# Autodesk Inventor assembly: cubi
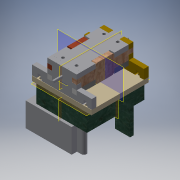
[picture p0: Inventor's stored thumbnail of the model, 180x180]
Saved by Autodesk Inventor 2018 (Build 220112000, 112)
## iProperties
Created: 2018-07-19
Part Number: cubi
Document SubType Name: Assembly
Designer: julien.allali
Author: julien.allali
## Documents named in this file (6)
- C:\Users\julien.allali\Documents\cubi\cubi.iam
- C:\Users\julien.allali\Documents\moteur.ipt
- C:\Users\julien.allali\Documents\cubi\board.ipt
- C:\Users\julien.allali\Documents\cubi\bat9V.ipt
- C:\Users\julien.allali\Documents\cubi\connector9V.ipt
- C:\Users\julien.allali\Documents\cubi\box.ipt
## Components (6 placed, 5 different names)
1. moteur:1 — Flush:1, Mate:1, Flush:2, Symmetry:1, Symmetry:2, Flush:5
2. moteur:2 — Flush:1, Mate:1, Flush:2, Mate:3, Symmetry:1, Symmetry:2, Flush:6
3. board:1 — Mate:2, Rotational:1, Mate:3, Mate:4, Mate:5, Flush:4, Flush:7
4. bat9V:1 — Flush:3, Mate:2
5. connector9V:1 — Flush:3, Rotational:1
6. box:1 — Flush:4, Flush:5, Flush:6, Flush:7
## Relationships (15: Flush 7, Mate 5, Symmetry 2, RevoluteJoint 1)
- Flush:1: moteur:1 ↔ moteur:2
- Mate:1 (5 mm): moteur:1 ↔ moteur:2
- Flush:2: moteur:1 ↔ moteur:2
- Flush:3: bat9V:1 ↔ connector9V:1
- Mate:2: board:1 ↔ bat9V:1
- Rotational:1 [RevoluteJoint] (-10 mm): board:1 ↔ connector9V:1
- Mate:3 (8 mm): moteur:2 ↔ board:1
- Symmetry:1: moteur:1 ↔ moteur:2
- Mate:4: board:1
- Symmetry:2: moteur:1 ↔ moteur:2
- Mate:5: board:1
- Flush:4: board:1 ↔ box:1
- Flush:5: moteur:1 ↔ box:1
- Flush:6: moteur:2 ↔ box:1
- Flush:7: board:1 ↔ box:1
